# Autodesk Inventor assembly: Motor
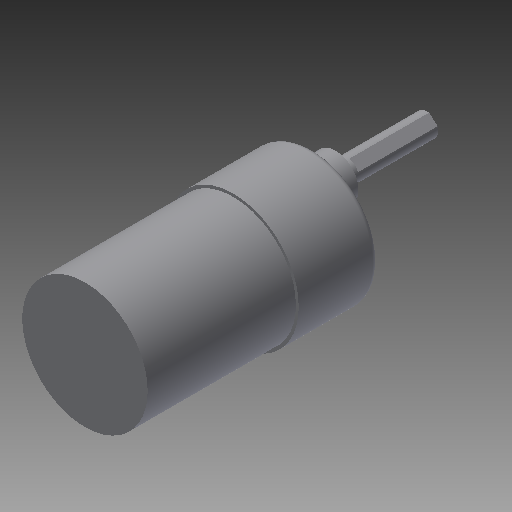
[picture p0: Inventor's stored thumbnail of the model, 512x512]
Saved by Autodesk Inventor 2017 (Build 210142000, 142)
## iProperties
Created: 2011-10-28
Part Number: Motor
Document SubType Name: Assembly
Designer: Kyle
Author: Kyle
## Documents named in this file (3)
- C:\Users\Spartacles\Desktop\FTC Parts\ftc-motor\Motor.iam
- C:\Users\Spartacles\Desktop\FTC Parts\ftc-motor\Motorbase.ipt
- C:\Users\Spartacles\Desktop\FTC Parts\ftc-motor\Motoraxle.ipt
## Components (2 placed, 2 different names)
1. Motorbase:1 — Mate:1, Tangent:1
2. Motoraxle:1 — Mate:1, Tangent:1
## Relationships (2: Mate 1, Tangent 1)
- Mate:1: Motorbase:1 ↔ Motoraxle:1
- Tangent:1: Motorbase:1 ↔ Motoraxle:1
